# Autodesk Inventor assembly: base_all
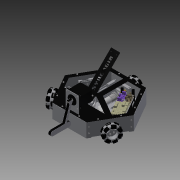
[picture p0: Inventor's stored thumbnail of the model, 180x180]
Saved by Autodesk Inventor 2015 (Build 190159000, 159)
## iProperties
Created: 2015-03-21
Part Number: base_all
Document SubType Name: Assembly
Designer: Marcin
Author: Marcin
## Documents named in this file (26)
- C:\Users\Kuba\Dysk Google\synergia\Synergolf\model\GOLF\base_all.iam
- C:\Users\Kuba\Dysk Google\synergia\Synergolf\model\GOLF\base_bottom.ipt
- C:\Users\Kuba\Dysk Google\synergia\Synergolf\model\GOLF\base_side.ipt
- C:\Users\Kuba\Dysk Google\synergia\Synergolf\model\GOLF\golf ball.ipt
- C:\Users\Kuba\Dysk Google\synergia\Synergolf\model\GOLF\base_const_al.iam
- C:\Users\Kuba\Dysk Google\synergia\Synergolf\model\GOLF\base_top.ipt
- C:\Users\Kuba\Dysk Google\synergia\Synergolf\model\GOLF\cover.ipt
- C:\Users\Kuba\Dysk Google\synergia\Synergolf\model\GOLF\martro_hettlich.iam
- C:\Users\Kuba\Dysk Google\synergia\Synergolf\model\GOLF\Połączenie gwintowe10.iam
- C:\Users\Kuba\Dysk Google\synergia\Synergolf\model\GOLF\base_side_constr.ipt
- C:\Users\Kuba\Dysk Google\synergia\Synergolf\model\GOLF\hinge_support.ipt
- C:\Users\Kuba\Dysk Google\synergia\Synergolf\model\GOLF\Połączenie gwintowe11.iam
- C:\Users\Kuba\Dysk Google\synergia\Synergolf\model\GOLF\Połączenie gwintowe12.iam
- C:\Users\Kuba\Dysk Google\synergia\Synergolf\model\GOLF\Połączenie gwintowe13.iam
- C:\Users\Kuba\Dysk Google\synergia\Synergolf\model\GOLF\Połączenie gwintowe14.iam
- C:\Users\Kuba\Dysk Google\synergia\Synergolf\model\GOLF\Połączenie gwintowe15.iam
- C:\Users\Kuba\Dysk Google\synergia\Synergolf\model\GOLF\Połączenie gwintowe16.iam
- C:\Users\Kuba\Dysk Google\synergia\Synergolf\model\GOLF\Połączenie gwintowe17.iam
- C:\Users\Kuba\Dysk Google\synergia\Synergolf\model\GOLF\Połączenie gwintowe18.iam
- C:\Users\Kuba\Dysk Google\synergia\Synergolf\model\GOLF\logo.ipt
- C:\Users\Kuba\Dysk Google\synergia\Synergolf\model\GOLF\Połączenie gwintowe19.iam
- C:\Users\Kuba\Dysk Google\synergia\Synergolf\model\GOLF\Połączenie gwintowe20.iam
- C:\Users\Kuba\Dysk Google\synergia\Synergolf\model\GOLF\Połączenie gwintowe21.iam
- C:\Users\Kuba\Dysk Google\synergia\Synergolf\model\GOLF\driver\motor driver support.iam
- C:\Users\Kuba\Dysk Google\synergia\Synergolf\model\GOLF\step driver support\step driver support.iam
- C:\Users\Kuba\Dysk Google\synergia\Synergolf\model\GOLF\batt support\batt support.iam
## Components (30 placed, 14 different names)
1. base_bottom:1 — Równoległy:1, Równoległy:2, Równoległy:3, Kąt:1, Zestawiający:13, Zestawiający:48, Zestawiający:49, Równoległy:25, Równoległy:26, Zestawiający:86, Zestawiający:87
2. golf ball:1 — Styczny:1
3. base_const_al:1 [sub-assembly] — Równoległy:16, Równoległy:17, Zestawiający:13, Zestawiający:59, Zestawiający:60, Zestawiający:64, Zestawiający:65, Zestawiający:89, Zestawiający:91, Zestawiający:94, Zestawiający:95, Zestawiający:96, Zestawiający:97
4. base_top:1 — Zestawiający:14, Zestawiający:15, Zestawiający:55, Zestawiający:58, Równoległy:28, Zestawiający:66, Zestawiający:67
5. cover:1 — Zestawiający:44, Zestawiający:63, Równoległy:29, Zestawiający:80, Równoległy:30
6. Połączenie gwintowe:8 [sub-assembly] — Zestawiający:48, Zestawiający:49
7. hinge_support:1 — Zestawiający:59, Równoległy:27, Zestawiający:60, Zestawiający:62
8. martro_hettlich:1 [sub-assembly] — Zestawiający:61, Zestawiający:62, Równoległy:28, Zestawiający:63, Równoległy:29
9. Połączenie gwintowe:9 [sub-assembly] — Zestawiający:64, Zestawiający:65
10. Połączenie gwintowe:10 [sub-assembly] — Zestawiający:66, Zestawiający:67
11. Połączenie gwintowe:11 [sub-assembly] — Zestawiający:68, Zestawiający:69
12. Połączenie gwintowe:12 [sub-assembly] — Zestawiający:70, Zestawiający:71
13. Połączenie gwintowe:13 [sub-assembly] — Zestawiający:72, Zestawiający:73
14. Połączenie gwintowe:14 [sub-assembly] — Zestawiający:74, Zestawiający:75
15. Połączenie gwintowe:15 [sub-assembly] — Zestawiający:76, Zestawiający:77
16. Połączenie gwintowe:16 [sub-assembly] — Zestawiający:78, Zestawiający:79
17. logo:1 — Zestawiający:80, Równoległy:30, Zestawiający:81, Zestawiający:82, Zestawiający:83, Zestawiający:84, Zestawiający:85
18. Połączenie gwintowe:17 [sub-assembly] — Zestawiający:82, Zestawiający:83
19. Połączenie gwintowe:18 [sub-assembly] — Zestawiający:84, Zestawiający:85
20. Połączenie gwintowe:19 [sub-assembly] — Zestawiający:86, Zestawiający:87
21. motor driver support:1 [sub-assembly] — Zestawiający:89, Zestawiający:94, Zestawiający:100
22. step driver support:1 [sub-assembly] — Zestawiający:91, Zestawiający:93, Zestawiający:99
23. motor driver support:2 [sub-assembly] — Zestawiający:95, Zestawiający:96, Zestawiający:101
24. batt support:1 [sub-assembly] — Zestawiający:97, Kąt:2, Zestawiający:98
25. base_side_constr:1 — Równoległy:25, Równoległy:26, Zestawiający:56, Zestawiający:101
26. base_side_constr:2 — Zestawiający:100
27. base_side_constr:3 — Zestawiający:55, Zestawiający:57
28. base_side:1 — Zestawiający:56, Zestawiający:57, Zestawiający:58, Zestawiający:68, Zestawiający:69, Zestawiający:70, Zestawiający:71
29. base_side:2 — Zestawiający:76, Zestawiający:77, Zestawiający:78, Zestawiający:79, Zestawiający:93
30. base_side:3 — Zestawiający:72, Zestawiający:73, Zestawiający:74, Zestawiający:75
## Component patterns: (3 elements, first: base_side_constr:1), (3 elements, first: base_side:1)
## Relationships (64: Mate 50, Flush 11, Angle 2, Tangent 1)
- Równoległy:1 [Flush]: base_bottom:1
- Równoległy:2 [Flush]: base_bottom:1
- Równoległy:3 [Flush]: base_bottom:1
- Kąt:1 [Angle] (0 deg): base_bottom:1
- Styczny:1 [Tangent]: golf ball:1
- Równoległy:16 [Flush]: base_const_al:1
- Równoległy:17 [Flush]: base_const_al:1
- Zestawiający:13 [Mate]: base_bottom:1 ↔ base_const_al:1
- Zestawiający:14 [Mate]: base_top:1
- Zestawiający:15 [Mate]: base_top:1
- Zestawiający:44 [Mate]: cover:1
- Zestawiający:48 [Mate]: base_bottom:1 ↔ Połączenie gwintowe:8
- Zestawiający:49 [Mate]: base_bottom:1 ↔ Połączenie gwintowe:8
- Równoległy:25 [Flush]: base_bottom:1 ↔ base_side_constr:1
- Równoległy:26 [Flush]: base_bottom:1 ↔ base_side_constr:1
- Zestawiający:55 [Mate]: base_top:1 ↔ base_side_constr:3
- Zestawiający:56 [Mate]: base_side_constr:1 ↔ base_side:1
- Zestawiający:57 [Mate]: base_side_constr:3 ↔ base_side:1
- Zestawiający:58 [Mate]: base_top:1 ↔ base_side:1
- Zestawiający:59 [Mate]: base_const_al:1 ↔ hinge_support:1
- Równoległy:27 [Flush]: hinge_support:1
- Zestawiający:60 [Mate]: base_const_al:1 ↔ hinge_support:1
- Zestawiający:61 [Mate]: martro_hettlich:1
- Zestawiający:62 [Mate]: hinge_support:1 ↔ martro_hettlich:1
- Równoległy:28 [Flush] (4.5 mm): base_top:1 ↔ martro_hettlich:1
- Zestawiający:63 [Mate]: cover:1 ↔ martro_hettlich:1
- Równoległy:29 [Flush] (-1.6 mm): cover:1 ↔ martro_hettlich:1
- Zestawiający:64 [Mate]: base_const_al:1 ↔ Połączenie gwintowe:9
- Zestawiający:65 [Mate]: base_const_al:1 ↔ Połączenie gwintowe:9
- Zestawiający:66 [Mate]: base_top:1 ↔ Połączenie gwintowe:10
- Zestawiający:67 [Mate]: base_top:1 ↔ Połączenie gwintowe:10
- Zestawiający:68 [Mate]: Połączenie gwintowe:11 ↔ base_side:1
- Zestawiający:69 [Mate]: Połączenie gwintowe:11 ↔ base_side:1
- Zestawiający:70 [Mate]: Połączenie gwintowe:12 ↔ base_side:1
- Zestawiający:71 [Mate]: Połączenie gwintowe:12 ↔ base_side:1
- Zestawiający:72 [Mate]: Połączenie gwintowe:13 ↔ base_side:3
- Zestawiający:73 [Mate]: Połączenie gwintowe:13 ↔ base_side:3
- Zestawiający:74 [Mate]: Połączenie gwintowe:14 ↔ base_side:3
- Zestawiający:75 [Mate]: Połączenie gwintowe:14 ↔ base_side:3
- Zestawiający:76 [Mate]: Połączenie gwintowe:15 ↔ base_side:2
- Zestawiający:77 [Mate]: Połączenie gwintowe:15 ↔ base_side:2
- Zestawiający:78 [Mate]: Połączenie gwintowe:16 ↔ base_side:2
- Zestawiający:79 [Mate]: Połączenie gwintowe:16 ↔ base_side:2
- Zestawiający:80 [Mate]: cover:1 ↔ logo:1
- Równoległy:30 [Flush] (1 mm): cover:1 ↔ logo:1
- Zestawiający:81 [Mate]: logo:1
- Zestawiający:82 [Mate]: logo:1 ↔ Połączenie gwintowe:17
- Zestawiający:83 [Mate]: logo:1 ↔ Połączenie gwintowe:17
- Zestawiający:84 [Mate]: logo:1 ↔ Połączenie gwintowe:18
- Zestawiający:85 [Mate]: logo:1 ↔ Połączenie gwintowe:18
- Zestawiający:86 [Mate]: base_bottom:1 ↔ Połączenie gwintowe:19
- Zestawiający:87 [Mate]: base_bottom:1 ↔ Połączenie gwintowe:19
- Zestawiający:89 [Mate]: base_const_al:1 ↔ motor driver support:1
- Zestawiający:91 [Mate]: base_const_al:1 ↔ step driver support:1
- Zestawiający:93 [Mate] (35 mm): step driver support:1 ↔ base_side:2
- Zestawiający:94 [Mate] (20 mm): base_const_al:1 ↔ motor driver support:1
- Zestawiający:95 [Mate] (20 mm): base_const_al:1 ↔ motor driver support:2
- Zestawiający:96 [Mate]: base_const_al:1 ↔ motor driver support:2
- Zestawiający:97 [Mate]: base_const_al:1 ↔ batt support:1
- Kąt:2 [Angle] (60 deg): batt support:1
- Zestawiający:98 [Mate]: batt support:1
- Zestawiający:99 [Mate]: step driver support:1
- Zestawiający:100 [Mate] (17 mm): motor driver support:1 ↔ base_side_constr:2
- Zestawiający:101 [Mate] (17 mm): motor driver support:2 ↔ base_side_constr:1
